# Autodesk Inventor assembly: Rev4StageSlider
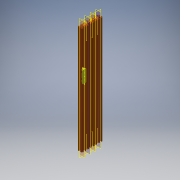
[picture p0: Inventor's stored thumbnail of the model, 180x180]
Saved by Autodesk Inventor 2018 (Build 220112000, 112)
## iProperties
Created: 2017-11-26
Part Number: Rev4StageSlider
Document SubType Name: Assembly
Designer: ball
Author: ball
## Documents named in this file (5)
- C:\FTC\FTC8863CAD\2017Robot\Rev4StageSlider.iam
- C:\FTC\FTC8863CAD\2017Robot\RevSingleStage.iam
- C:\FTC\FTC8863CAD\RevRobotics\REV-41-1039.ipt
- C:\FTC\FTC8863CAD\RevRobotics\REV-41-1094.ipt
- C:\FTC\FTC8863CAD\RevRobotics\REV-41-1095.ipt
## Components (10 placed, 4 different names)
1. RevSingleStage:1 [sub-assembly] — Mate:1, Flush:1, Flush:15, Flush:17, Flush:18, Mate:7, Flush:19, Flush:20, Mate:8, Flush:21, Flush:22, Flush:27, Mate:12, Mate:13
2. RevSingleStage:2 [sub-assembly] — Mate:1, Flush:1, Flush:15
3. RevSingleStage:8 [sub-assembly] — Flush:14
4. RevSingleStage:9 [sub-assembly] — Flush:14, Flush:21, Flush:22, Mate:9, Flush:28, Flush:29, Mate:14
5. REV-41-1094:2 — Flush:19, Flush:20, Mate:8, Mate:9
6. REV-41-1094:3 — Flush:17, Flush:18, Mate:7, Flush:31
7. REV-41-1095:6 — Flush:28, Flush:29, Mate:14, Flush:30, Mate:15
8. REV-41-1095:7 — Flush:27, Mate:12, Mate:13
9. REV-41-1039:5 — Flush:30, Flush:31, Mate:15
10. REV-41-1095:8
## Relationships (24: Flush 15, Mate 9)
- Mate:1: RevSingleStage:1 ↔ RevSingleStage:2
- Flush:1: RevSingleStage:1 ↔ RevSingleStage:2
- [Mate]: RevSingleStage:8 ↔ RevSingleStage:9
- [Flush]: RevSingleStage:8 ↔ RevSingleStage:9
- Flush:14: RevSingleStage:8 ↔ RevSingleStage:9
- Flush:15: RevSingleStage:1 ↔ RevSingleStage:2
- Flush:17: RevSingleStage:1 ↔ REV-41-1094:3
- Flush:18: RevSingleStage:1 ↔ REV-41-1094:3
- Mate:7: RevSingleStage:1 ↔ REV-41-1094:3
- Flush:19: RevSingleStage:1 ↔ REV-41-1094:2
- Flush:20: RevSingleStage:1 ↔ REV-41-1094:2
- Mate:8: RevSingleStage:1 ↔ REV-41-1094:2
- Flush:21: RevSingleStage:1 ↔ RevSingleStage:9
- Flush:22: RevSingleStage:1 ↔ RevSingleStage:9
- Mate:9: RevSingleStage:9 ↔ REV-41-1094:2
- Flush:27: RevSingleStage:1 ↔ REV-41-1095:7
- Flush:28: RevSingleStage:9 ↔ REV-41-1095:6
- Mate:12: RevSingleStage:1 ↔ REV-41-1095:7
- Mate:13: RevSingleStage:1 ↔ REV-41-1095:7
- Flush:29: RevSingleStage:9 ↔ REV-41-1095:6
- Mate:14: RevSingleStage:9 ↔ REV-41-1095:6
- Flush:30: REV-41-1095:6 ↔ REV-41-1039:5
- Flush:31: REV-41-1094:3 ↔ REV-41-1039:5
- Mate:15: REV-41-1095:6 ↔ REV-41-1039:5
## Named parameters: d12_d1 = 0 mm, d13_d2 = 0 mm
